# Autodesk Inventor assembly: oikon
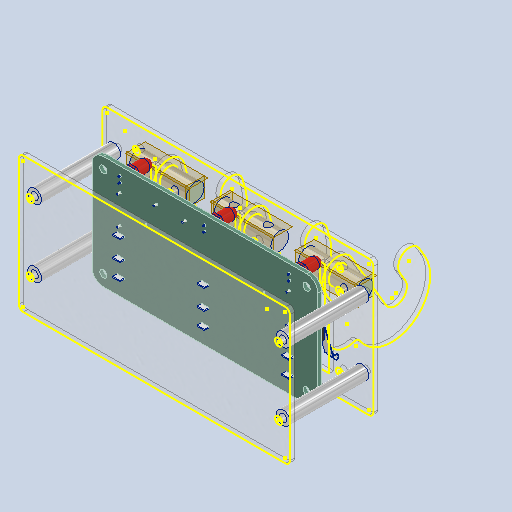
[picture p0: Inventor's stored thumbnail of the model, 512x512]
Saved by Autodesk Inventor 2025.2 (Build 292293000, 293)
## iProperties
Created: 2025-02-28
Part Number: oikon
Document SubType Name: Assembly
Designer: haruy
Author: haruy
## Documents named in this file (7)
- C:\Users\haruy\Documents\ロボコン\NHK2025\cad\nagahisa\oikon\oikon.iam
- C:\Users\haruy\Documents\ロボコン\NHK2025\cad\nagahisa\oikon\part1.ipt
- C:\Users\haruy\Documents\ロボコン\NHK2025\cad\nagahisa\oikon\part2.ipt
- C:\Users\haruy\Documents\ロボコン\NHK2025\cad\nagahisa\oikon\part3.ipt
- C:\Users\haruy\Documents\ロボコン\NHK2025\cad\nagahisa\oikon\part4.ipt
- C:\Users\haruy\Documents\ロボコン\NHK2025\cad\nagahisa\oikon\part6.ipt
- C:\Users\haruy\Documents\ロボコン\NHK2025\cad\nagahisa\oikon\part7.ipt
## Components (13 placed, 6 different names)
1. part1:1 — メイト:1, メイト:2, フラッシュ:1, メイト:3, フラッシュ:2, フラッシュ:3, フラッシュ:4, メイト:4, 挿入:10, 挿入:11, 挿入:16
2. part2:1 — メイト:1, メイト:2, フラッシュ:2, メイト:5, 挿入:1
3. part2:2 — フラッシュ:4, メイト:4, メイト:5, 挿入:2
4. part2:3 — フラッシュ:1, メイト:3, フラッシュ:3, 挿入:3
5. part3:1 — 挿入:1
6. part3:2 — 挿入:2
7. part3:3 — 挿入:3
8. part4:1 — 挿入:14, 挿入:15
9. part6:1 — 挿入:10, 挿入:14
10. part6:2 — 挿入:11, 挿入:15
11. part6:3
12. part6:4
13. part7:1 — 挿入:16
## Relationships (17: Insert 8, Mate 5, Flush 4)
- メイト:1 [Mate] (-10 mm): part1:1 ↔ part2:1
- メイト:2 [Mate]: part1:1 ↔ part2:1
- フラッシュ:1 [Flush] (10 mm): part1:1 ↔ part2:3
- メイト:3 [Mate]: part1:1 ↔ part2:3
- フラッシュ:2 [Flush] (15 mm): part1:1 ↔ part2:1
- フラッシュ:3 [Flush] (15 mm): part1:1 ↔ part2:3
- フラッシュ:4 [Flush] (15 mm): part1:1 ↔ part2:2
- メイト:4 [Mate]: part1:1 ↔ part2:2
- メイト:5 [Mate] (12.2 mm): part2:1 ↔ part2:2
- 挿入:1 [Insert] (-11.6 mm): part2:1 ↔ part3:1
- 挿入:2 [Insert] (11.6 mm): part2:2 ↔ part3:2
- 挿入:3 [Insert] (11.6 mm): part2:3 ↔ part3:3
- 挿入:10 [Insert]: part1:1 ↔ part6:1
- 挿入:11 [Insert]: part1:1 ↔ part6:2
- 挿入:14 [Insert]: part4:1 ↔ part6:1
- 挿入:15 [Insert]: part4:1 ↔ part6:2
- 挿入:16 [Insert] (13 mm): part1:1 ↔ part7:1
